# Autodesk Inventor assembly: hand
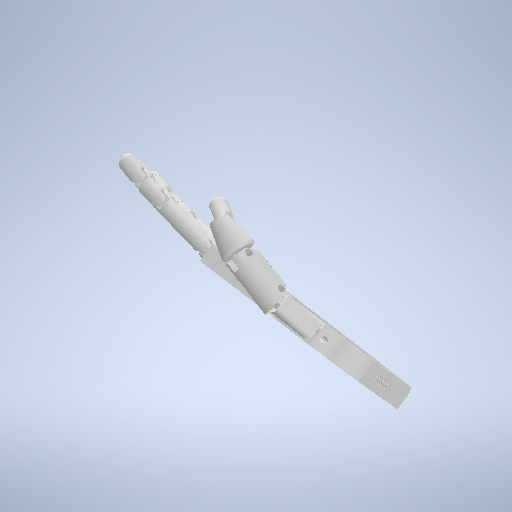
[picture p0: Inventor's stored thumbnail of the model, 512x512]
Saved by Autodesk Inventor 2025 (Build 290162000, 162)
## iProperties
Created: 2025-10-18
Part Number: hand
Document SubType Name: Assembly
Designer: abdul
Author: abdul
## Documents named in this file (24)
- C:\Users\abdul\OneDrive\Documents\Prosthetic hand\idea 2\hand.iam
- C:\Users\abdul\OneDrive\Documents\Prosthetic hand\idea 2\Pinky\PART 2 OF FINGER(pinky).ipt
- C:\Users\abdul\OneDrive\Documents\Prosthetic hand\idea 2\Pinky\Part1 finger tip(pinky).ipt
- C:\Users\abdul\OneDrive\Documents\Prosthetic hand\idea 2\Pinky\Part3 of finger(pinky).ipt
- C:\Users\abdul\OneDrive\Documents\Prosthetic hand\idea 2\Pinky\Part4 finger(pinky).ipt
- C:\Users\abdul\OneDrive\Documents\Prosthetic hand\idea 2\joint.ipt
- C:\Users\abdul\OneDrive\Documents\Prosthetic hand\idea 2\ring\PART 2 OF FINGER(ring).ipt
- C:\Users\abdul\OneDrive\Documents\Prosthetic hand\idea 2\ring\Part1 finger tip(ring).ipt
- C:\Users\abdul\OneDrive\Documents\Prosthetic hand\idea 2\ring\Part3 of finger(ring).ipt
- C:\Users\abdul\OneDrive\Documents\Prosthetic hand\idea 2\ring\Part4 finger(ring).ipt
- C:\Users\abdul\OneDrive\Documents\Prosthetic hand\idea 2\middle\PART 2 OF FINGER(middle).ipt
- C:\Users\abdul\OneDrive\Documents\Prosthetic hand\idea 2\middle\Part1 finger tip(middle).ipt
- C:\Users\abdul\OneDrive\Documents\Prosthetic hand\idea 2\middle\Part3 of finger(middle).ipt
- C:\Users\abdul\OneDrive\Documents\Prosthetic hand\idea 2\middle\Part4 finger(middle).ipt
- C:\Users\abdul\OneDrive\Documents\Prosthetic hand\idea 2\index\PART 2 OF FINGER(index).ipt
- C:\Users\abdul\OneDrive\Documents\Prosthetic hand\idea 2\index\Part1 finger tip(indeex).ipt
- C:\Users\abdul\OneDrive\Documents\Prosthetic hand\idea 2\index\Part3 of finger(index).ipt
- C:\Users\abdul\OneDrive\Documents\Prosthetic hand\idea 2\index\Part4 finger(index).ipt
- C:\Users\abdul\OneDrive\Documents\Prosthetic hand\idea 2\main hand.ipt
- C:\Users\abdul\OneDrive\Documents\Prosthetic hand\idea 2\thumb 1st part (model 2).ipt
- C:\Users\abdul\OneDrive\Documents\Prosthetic hand\idea 2\thumb 4th part (model 2).ipt
- C:\Users\abdul\OneDrive\Documents\Prosthetic hand\idea 2\thumb 5th part (model 2).ipt
- C:\Users\abdul\OneDrive\Documents\Prosthetic hand\idea 2\thumb 6th part(model 2).ipt
- C:\Users\abdul\OneDrive\Documents\Prosthetic hand\idea 2\thumb base((model 2).ipt
## Components (36 placed, 23 different names)
1. PART 2 OF FINGER(pinky):1 — Rigid:2, Insert:7, Insert:8
2. Part1 finger tip(pinky):1 — Rigid:5
3. Part3 of finger(pinky):1 — Rigid:2, Insert:3, Insert:4
4. Part4 finger(pinky):1 — Insert:3, Rigid:10
5. Part3 of finger(pinky):2 — Insert:7, Rigid:5
6. joint:1 — Insert:8
7. joint:2 — Insert:4
8. PART 2 OF FINGER(ring):1 — Rigid:4, Insert:5
9. Part1 finger tip(ring):1 — Rigid:3
10. Part3 of finger(ring):1 — Rigid:3, Insert:5
11. Part4 finger(ring):1 — Insert:6, Rigid:11
12. Part3 of finger(ring):2 — Rigid:4, Insert:6
13. joint:3 — Insert:12
14. joint:4 — Insert:11
15. joint:5 — Insert:15
16. joint:6 — Insert:16
17. Part1 finger tip(middle):1 — Rigid:8
18. Part3 of finger(middle):1 — Rigid:8, Insert:13, Insert:15
19. Part4 finger(middle):1 — Insert:14, Rigid:12
20. PART 2 OF FINGER(middle):2 — Rigid:9, Insert:13
21. Part3 of finger(middle):2 — Rigid:9, Insert:14, Insert:16
22. PART 2 OF FINGER(index):1 — Rigid:7, Insert:9
23. Part1 finger tip(indeex):1 — Rigid:6
24. Part3 of finger(index):1 — Rigid:6, Insert:9, Insert:11
25. Part4 finger(index):1 — Insert:10, Rigid:13
26. Part3 of finger(index):2 — Rigid:7, Insert:10, Insert:12
27. Part3 of finger(pinky):3 — Rigid:10, Rotational:4
28. Part3 of finger(ring):3 — Rigid:11, Rotational:3
29. Part3 of finger(middle):3 — Rigid:12, Rotational:2
30. Part3 of finger(index):3 — Rigid:13, Rotational:8
31. main hand:1 — Rotational:2, Rotational:3, Rotational:4, Rotational:7, Rotational:8
32. thumb 1st part (model 2):1 — Rigid:15, Rotational:6
33. thumb 4th part (model 2):1 — Rigid:14, Rigid:15
34. thumb 5th part (model 2):1 — Rigid:14, Rotational:5
35. thumb 6th part(model 2):1 — Rotational:5
36. thumb base((model 2):1 — Rotational:6, Rotational:7
## Relationships (35: WeldJoint 14, Insert 14, RevoluteJoint 7)
- Rigid:2 [WeldJoint]: PART 2 OF FINGER(pinky):1 ↔ Part3 of finger(pinky):1
- Insert:3 (0.3 mm): Part3 of finger(pinky):1 ↔ Part4 finger(pinky):1
- Insert:4 (-1.8 mm): Part3 of finger(pinky):1 ↔ joint:2
- Rigid:3 [WeldJoint]: Part1 finger tip(ring):1 ↔ Part3 of finger(ring):1
- Rigid:4 [WeldJoint]: PART 2 OF FINGER(ring):1 ↔ Part3 of finger(ring):2
- Insert:5 (0.3 mm): PART 2 OF FINGER(ring):1 ↔ Part3 of finger(ring):1
- Insert:6: Part4 finger(ring):1 ↔ Part3 of finger(ring):2
- Insert:7 (0.3 mm): PART 2 OF FINGER(pinky):1 ↔ Part3 of finger(pinky):2
- Insert:8 (-2.1 mm): PART 2 OF FINGER(pinky):1 ↔ joint:1
- Rigid:5 [WeldJoint]: Part1 finger tip(pinky):1 ↔ Part3 of finger(pinky):2
- Rigid:6 [WeldJoint]: Part1 finger tip(indeex):1 ↔ Part3 of finger(index):1
- Rigid:7 [WeldJoint]: PART 2 OF FINGER(index):1 ↔ Part3 of finger(index):2
- Insert:9 (0.3 mm): PART 2 OF FINGER(index):1 ↔ Part3 of finger(index):1
- Insert:10 (0.3 mm): Part4 finger(index):1 ↔ Part3 of finger(index):2
- Insert:11 (-1.8 mm): joint:4 ↔ Part3 of finger(index):1
- Insert:12 (-1.8 mm): joint:3 ↔ Part3 of finger(index):2
- Rigid:8 [WeldJoint]: Part1 finger tip(middle):1 ↔ Part3 of finger(middle):1
- Rigid:9 [WeldJoint]: PART 2 OF FINGER(middle):2 ↔ Part3 of finger(middle):2
- Insert:13 (0.3 mm): Part3 of finger(middle):1 ↔ PART 2 OF FINGER(middle):2
- Insert:14 (0.3 mm): Part4 finger(middle):1 ↔ Part3 of finger(middle):2
- Insert:15 (-1.8 mm): joint:5 ↔ Part3 of finger(middle):1
- Insert:16 (-1.8 mm): joint:6 ↔ Part3 of finger(middle):2
- Rigid:10 [WeldJoint]: Part4 finger(pinky):1 ↔ Part3 of finger(pinky):3
- Rigid:11 [WeldJoint]: Part4 finger(ring):1 ↔ Part3 of finger(ring):3
- Rigid:12 [WeldJoint]: Part4 finger(middle):1 ↔ Part3 of finger(middle):3
- Rigid:13 [WeldJoint]: Part4 finger(index):1 ↔ Part3 of finger(index):3
- Rotational:2 [RevoluteJoint]: Part3 of finger(middle):3 ↔ main hand:1
- Rotational:3 [RevoluteJoint]: Part3 of finger(ring):3 ↔ main hand:1
- Rotational:4 [RevoluteJoint]: Part3 of finger(pinky):3 ↔ main hand:1
- Rigid:14 [WeldJoint]: thumb 4th part (model 2):1 ↔ thumb 5th part (model 2):1
- Rigid:15 [WeldJoint]: thumb 1st part (model 2):1 ↔ thumb 4th part (model 2):1
- Rotational:5 [RevoluteJoint]: thumb 5th part (model 2):1 ↔ thumb 6th part(model 2):1
- Rotational:6 [RevoluteJoint]: thumb 1st part (model 2):1 ↔ thumb base((model 2):1
- Rotational:7 [RevoluteJoint] (0.5 mm): main hand:1 ↔ thumb base((model 2):1
- Rotational:8 [RevoluteJoint]: Part3 of finger(index):3 ↔ main hand:1
